# Autodesk Inventor assembly: ASY MSC 800 gills
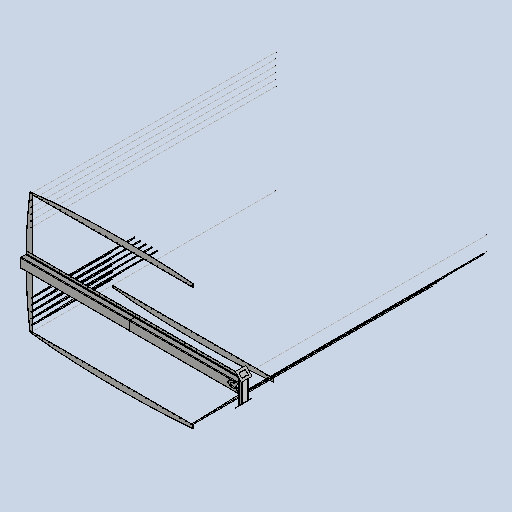
[picture p0: Inventor's stored thumbnail of the model, 512x512]
Saved by Autodesk Inventor 2025 (Build 290162010, 162A)
## iProperties
Created: 2024-08-31
Part Number: ASY MSC 800 gills
Document SubType Name: Assembly
Designer: pokla
Stock Number: ASY МОО 800 Жабры
Mass: 57918.9 g
Surface Area: 154099 cm^2
Volume: 7985.94 cm^3
Density: 7.25262 g/cm^3
Author: pokla
## Documents named in this file (15)
- C:\Users\admin\YandexDisk-badmisterfox\домашниий пк\Inventor\Manturovo\Manturovo_Se-clar\ASY MSC 080 gills.iam
- C:\Users\admin\YandexDisk-badmisterfox\домашниий пк\Inventor\Manturovo\Manturovo_Se-clar\MSC 802 sheet gills.ipt
- C:\Users\admin\YandexDisk-badmisterfox\домашниий пк\Inventor\Manturovo\Manturovo_Se-clar\MSC 081 pillar gills.ipt
- C:\Users\admin\YandexDisk-badmisterfox\домашниий пк\Inventor\Manturovo\Manturovo_Se-clar\MSC 803 sheet gills.ipt
- C:\Users\admin\YandexDisk-badmisterfox\домашниий пк\Inventor\Manturovo\Manturovo_Se-clar\MSC 805 sheet gills.ipt
- C:\Users\admin\YandexDisk-badmisterfox\домашниий пк\Inventor\Manturovo\Manturovo_Se-clar\MSC 807 sheet gills.ipt
- C:\Users\admin\YandexDisk-badmisterfox\домашниий пк\Inventor\Manturovo\Manturovo_Se-clar\MSC 809 sheet gills.ipt
- C:\Users\admin\YandexDisk-badmisterfox\домашниий пк\Inventor\Manturovo\Manturovo_Se-clar\MSC 811 sheet gills.ipt
- C:\Users\admin\YandexDisk-badmisterfox\домашниий пк\Inventor\Manturovo\Manturovo_Se-clar\MSC 084 wall support gills.ipt
- C:\Users\admin\YandexDisk-badmisterfox\домашниий пк\Inventor\Manturovo\Manturovo_Se-clar\MSC 082 pillar gills.ipt
- C:\Users\admin\YandexDisk-badmisterfox\домашниий пк\Inventor\Manturovo\Manturovo_Se-clar\MSC 086 string for sheets gills.ipt
- C:\Users\admin\YandexDisk-badmisterfox\домашниий пк\Inventor\Manturovo\Manturovo_Se-clar\MSC 083 top support gills.ipt
- C:\Users\admin\YandexDisk-badmisterfox\домашниий пк\Inventor\Manturovo\Manturovo_Se-clar\MSC 801 sheet gills.ipt
- C:\Users\admin\YandexDisk-badmisterfox\домашниий пк\Inventor\Manturovo\Manturovo_Se-clar\ASY MSC 089 gills base.iam
- C:\Users\admin\YandexDisk-badmisterfox\домашниий пк\Inventor\Manturovo\Manturovo_Se-clar\MSC 082 pillar 2.ipt
## Components (26 placed, 14 different names)
1. MSC 803 sheet gills.ipt:1 — Angle:2, Tangent:8, Tangent:9, Flush:15, Flush:19
2. MSC 805 sheet gills.ipt:1 — Angle:3, Tangent:10, Tangent:11, Flush:15, Flush:16
3. MSC 807 sheet gills.ipt:1 — Angle:4, Tangent:12, Tangent:13, Flush:16, Flush:17
4. MSC 809 sheet gills.ipt:1 — Angle:5, Tangent:17, Tangent:18, Flush:17, Flush:18
5. MSC 811 sheet gills.ipt:1 — Angle:6, Tangent:19, Tangent:20, Flush:18
6. MSC 084 wall support gills.ipt:1 — Rigid:12, Rigid:25, Rigid:30, Tangent:14, Tangent:15
7. MSC 084 wall support gills.ipt:2 — Rigid:25, Mate:17
8. MSC 084 wall support gills.ipt:3 — Rigid:31
9. MSC 083 top support gills.ipt:2 — Rigid:28, Rigid:30, Tangent:8, Tangent:9, Tangent:10, Tangent:11, Tangent:12, Tangent:13, Tangent:17, Tangent:18, Tangent:19, Tangent:20, Rigid:40
10. MSC 083 top support gills.ipt:1 — Rigid:24, Rigid:29, Rigid:31
11. ASY MSC 089 gills base.iam:1 [sub-assembly]
12. MSC 082 pillar gills.ipt:1 — Rigid:28, Rigid:29
13. MSC 081 pillar gills.ipt:1 — Rotational:1, Rotational:2, Tangent:16, Mate:18
14. MSC 802 sheet gills.ipt:1 — Rigid:33
15. MSC 801 sheet gills.ipt:1 — Mate:17, Rigid:33, Angle:2, Angle:3, Angle:4, Angle:5, Angle:6, Tangent:14, Tangent:15, Tangent:16, Flush:19
16. MSC 086 string for sheets gills.ipt:1 — Rigid:12
17. MSC 082 pillar 2.ipt:1 — Mate:18
18. MSC 086 string for sheets gills.ipt:3 — Rotational:2
19. MSC 086 string for sheets gills.ipt:2 — Rotational:1
20. MSC 086 string for sheets gills.ipt:4 — Rigid:40
21. MSC 086 string for sheets gills.ipt:5 — Rigid:24
22. MSC 086 string for sheets gills.ipt:6
23. MSC 086 string for sheets gills.ipt:7
24. MSC 086 string for sheets gills.ipt:8
25. MSC 086 string for sheets gills.ipt:9
26. MSC 086 string for sheets gills.ipt:10
## Component patterns: (6 elements, first: MSC 086 string for sheets gills.ipt:5)
## Relationships (43: Tangent 13, WeldJoint 10, Flush 8, Mate 5, Angle 5, RevoluteJoint 2)
- [WeldJoint]: MSC 082 pillar gills.ipt:1 ↔ MSC 081 pillar gills.ipt:1
- [Flush]: ASY MSC 089 gills base.iam:1 ↔ MSC 081 pillar gills.ipt:1
- [Mate]: ASY MSC 089 gills base.iam:1 ↔ MSC 081 pillar gills.ipt:1
- [Flush] (5 mm): ASY MSC 089 gills base.iam:1 ↔ MSC 081 pillar gills.ipt:1
- Rigid:12 [WeldJoint] (-5 mm): MSC 084 wall support gills.ipt:1 ↔ MSC 086 string for sheets gills.ipt:1
- [Mate]: ASY MSC 089 gills base.iam:1
- [Mate]: ASY MSC 089 gills base.iam:1
- [Flush]: ASY MSC 089 gills base.iam:1
- Rigid:24 [WeldJoint] (-5 mm): MSC 083 top support gills.ipt:1 ↔ MSC 086 string for sheets gills.ipt:5
- Rigid:25 [WeldJoint] (985 mm): MSC 084 wall support gills.ipt:1 ↔ MSC 084 wall support gills.ipt:2
- Mate:17: MSC 084 wall support gills.ipt:2 ↔ MSC 801 sheet gills.ipt:1
- Rigid:28 [WeldJoint]: MSC 083 top support gills.ipt:2 ↔ MSC 082 pillar gills.ipt:1
- Rigid:29 [WeldJoint]: MSC 083 top support gills.ipt:1 ↔ MSC 082 pillar gills.ipt:1
- Rigid:30 [WeldJoint]: MSC 084 wall support gills.ipt:1 ↔ MSC 083 top support gills.ipt:2
- Rigid:31 [WeldJoint]: MSC 084 wall support gills.ipt:3 ↔ MSC 083 top support gills.ipt:1
- Rotational:1 [RevoluteJoint] (5 mm): MSC 081 pillar gills.ipt:1 ↔ MSC 086 string for sheets gills.ipt:2
- Rotational:2 [RevoluteJoint] (-5 mm): MSC 081 pillar gills.ipt:1 ↔ MSC 086 string for sheets gills.ipt:3
- Rigid:33 [WeldJoint] (-10 mm): MSC 802 sheet gills.ipt:1 ↔ MSC 801 sheet gills.ipt:1
- Angle:2 (0 deg): MSC 803 sheet gills.ipt:1 ↔ MSC 801 sheet gills.ipt:1
- Angle:3 (0 deg): MSC 805 sheet gills.ipt:1 ↔ MSC 801 sheet gills.ipt:1
- Angle:4 (0 deg): MSC 807 sheet gills.ipt:1 ↔ MSC 801 sheet gills.ipt:1
- Angle:5 (0 deg): MSC 809 sheet gills.ipt:1 ↔ MSC 801 sheet gills.ipt:1
- Angle:6 (0 deg): MSC 811 sheet gills.ipt:1 ↔ MSC 801 sheet gills.ipt:1
- Tangent:8: MSC 803 sheet gills.ipt:1 ↔ MSC 083 top support gills.ipt:2
- Tangent:9: MSC 803 sheet gills.ipt:1 ↔ MSC 083 top support gills.ipt:2
- Tangent:10: MSC 805 sheet gills.ipt:1 ↔ MSC 083 top support gills.ipt:2
- Tangent:11: MSC 805 sheet gills.ipt:1 ↔ MSC 083 top support gills.ipt:2
- Tangent:12: MSC 807 sheet gills.ipt:1 ↔ MSC 083 top support gills.ipt:2
- Tangent:13: MSC 807 sheet gills.ipt:1 ↔ MSC 083 top support gills.ipt:2
- Tangent:14: MSC 084 wall support gills.ipt:1 ↔ MSC 801 sheet gills.ipt:1
- Tangent:15: MSC 084 wall support gills.ipt:1 ↔ MSC 801 sheet gills.ipt:1
- Tangent:16: MSC 081 pillar gills.ipt:1 ↔ MSC 801 sheet gills.ipt:1
- Tangent:17: MSC 809 sheet gills.ipt:1 ↔ MSC 083 top support gills.ipt:2
- Tangent:18: MSC 809 sheet gills.ipt:1 ↔ MSC 083 top support gills.ipt:2
- Tangent:19: MSC 811 sheet gills.ipt:1 ↔ MSC 083 top support gills.ipt:2
- Tangent:20: MSC 811 sheet gills.ipt:1 ↔ MSC 083 top support gills.ipt:2
- Flush:15: MSC 803 sheet gills.ipt:1 ↔ MSC 805 sheet gills.ipt:1
- Flush:16: MSC 805 sheet gills.ipt:1 ↔ MSC 807 sheet gills.ipt:1
- Flush:17: MSC 807 sheet gills.ipt:1 ↔ MSC 809 sheet gills.ipt:1
- Flush:18: MSC 809 sheet gills.ipt:1 ↔ MSC 811 sheet gills.ipt:1
- Flush:19: MSC 803 sheet gills.ipt:1 ↔ MSC 801 sheet gills.ipt:1
- Rigid:40 [WeldJoint] (5 mm): MSC 083 top support gills.ipt:2 ↔ MSC 086 string for sheets gills.ipt:4
- Mate:18: MSC 081 pillar gills.ipt:1 ↔ MSC 082 pillar 2.ipt:1
